# Autodesk Inventor assembly: modeloRaspi
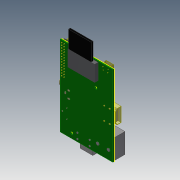
[picture p0: Inventor's stored thumbnail of the model, 180x180]
Saved by Autodesk Inventor 2014 (Build 180170000, 170)
## iProperties
Created: 2013-09-17
Part Number: modeloRaspi
Document SubType Name: Assembly
Designer: Eden
Author: Eden
## Documents named in this file (10)
- C:\Users\Eden\Documents\Inventor\raspiCase\modeloRaspi.iam
- C:\Users\Eden\Documents\Inventor\raspiCase\baseRaspi.ipt
- C:\Users\Eden\Documents\Inventor\raspiCase\conMiniUSB.ipt
- C:\Users\Eden\Documents\Inventor\raspiCase\conHDMI.ipt
- C:\Users\Eden\Documents\Inventor\raspiCase\conRJ45.ipt
- C:\Users\Eden\Documents\Inventor\raspiCase\conUSBA.ipt
- C:\Users\Eden\Documents\Inventor\raspiCase\con35mm.ipt
- C:\Users\Eden\Documents\Inventor\raspiCase\conRCA.ipt
- C:\Users\Eden\Documents\Inventor\raspiCase\pin254.iam
- C:\Users\Eden\Documents\Inventor\raspiCase\conSD.ipt
## Components (21 placed, 9 different names)
1. baseRaspi:1 — Mate:1, Mate:2, Mate:3, Mate:4, Mate:5, Mate:6, Mate:7, Mate:8, Mate:9, Mate:10, Mate:11, Mate:12, Mate:13, Mate:14, Mate:15, Mate:16, Mate:17, Mate:18, Rigid:1, Rigid:2, Rigid:3, Rigid:4, Rigid:5, Rigid:6, Rigid:7, Rigid:8, Rigid:9, Rigid:10, Rigid:11, Rigid:12, Rigid:13, Mate:19, Mate:20, Mate:21
2. conMiniUSB:1 — Mate:1, Mate:2, Mate:3
3. conHDMI:1 — Mate:4, Mate:5, Mate:6
4. conRJ45:1 — Mate:7, Mate:8, Mate:9
5. conUSBA:1 — Mate:10, Mate:11, Mate:12, Mate:13
6. con35mm:1 — Mate:14, Mate:15, Mate:16
7. conRCA:1 — Mate:17, Mate:18
8. pin254:1 [sub-assembly] — Rigid:1
9. pin254:2 [sub-assembly] — Rigid:10
10. pin254:3 [sub-assembly] — Rigid:11
11. pin254:4 [sub-assembly] — Rigid:12
12. pin254:5 [sub-assembly] — Rigid:3
13. pin254:6 [sub-assembly] — Rigid:6
14. pin254:7 [sub-assembly] — Rigid:8
15. pin254:8 [sub-assembly] — Rigid:7
16. pin254:9 [sub-assembly] — Rigid:13
17. pin254:10 [sub-assembly] — Rigid:2
18. pin254:11 [sub-assembly] — Rigid:4
19. pin254:12 [sub-assembly] — Rigid:5
20. pin254:13 [sub-assembly] — Rigid:9
21. conSD:1 — Mate:19, Mate:20, Mate:21
## Relationships (34: Mate 21, WeldJoint 13)
- Mate:1: baseRaspi:1 ↔ conMiniUSB:1
- Mate:2: baseRaspi:1 ↔ conMiniUSB:1
- Mate:3: baseRaspi:1 ↔ conMiniUSB:1
- Mate:4: baseRaspi:1 ↔ conHDMI:1
- Mate:5: baseRaspi:1 ↔ conHDMI:1
- Mate:6: baseRaspi:1 ↔ conHDMI:1
- Mate:7: baseRaspi:1 ↔ conRJ45:1
- Mate:8: baseRaspi:1 ↔ conRJ45:1
- Mate:9: baseRaspi:1 ↔ conRJ45:1
- Mate:10: baseRaspi:1 ↔ conUSBA:1
- Mate:11: baseRaspi:1 ↔ conUSBA:1
- Mate:12: baseRaspi:1 ↔ conUSBA:1
- Mate:13: baseRaspi:1 ↔ conUSBA:1
- Mate:14: baseRaspi:1 ↔ con35mm:1
- Mate:15: baseRaspi:1 ↔ con35mm:1
- Mate:16: baseRaspi:1 ↔ con35mm:1
- Mate:17: baseRaspi:1 ↔ conRCA:1
- Mate:18: baseRaspi:1 ↔ conRCA:1
- Rigid:1 [WeldJoint] (2.45 mm): baseRaspi:1 ↔ pin254:1
- Rigid:2 [WeldJoint] (-0.95 mm): baseRaspi:1 ↔ pin254:10
- Rigid:3 [WeldJoint] (-0.95 mm): baseRaspi:1 ↔ pin254:5
- Rigid:4 [WeldJoint] (-0.95 mm): baseRaspi:1 ↔ pin254:11
- Rigid:5 [WeldJoint] (-0.95 mm): baseRaspi:1 ↔ pin254:12
- Rigid:6 [WeldJoint] (-0.95 mm): baseRaspi:1 ↔ pin254:6
- Rigid:7 [WeldJoint] (-0.95 mm): baseRaspi:1 ↔ pin254:8
- Rigid:8 [WeldJoint] (-0.95 mm): baseRaspi:1 ↔ pin254:7
- Rigid:9 [WeldJoint] (-0.95 mm): baseRaspi:1 ↔ pin254:13
- Rigid:10 [WeldJoint] (-0.95 mm): baseRaspi:1 ↔ pin254:2
- Rigid:11 [WeldJoint] (-0.95 mm): baseRaspi:1 ↔ pin254:3
- Rigid:12 [WeldJoint] (-0.95 mm): baseRaspi:1 ↔ pin254:4
- Rigid:13 [WeldJoint] (-0.95 mm): baseRaspi:1 ↔ pin254:9
- Mate:19: baseRaspi:1 ↔ conSD:1
- Mate:20 (12 mm): baseRaspi:1 ↔ conSD:1
- Mate:21 (1 mm): baseRaspi:1 ↔ conSD:1
